(part 1 of 2)
# Autodesk Inventor assembly: enix_assembly_v2
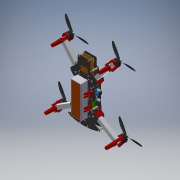
[picture p0: Inventor's stored thumbnail of the model, 180x180]
Saved by Autodesk Inventor 2016 (Build 200138000, 138)
## iProperties
Created: 2016-09-22
Part Number: enix_assembly_v2
Document SubType Name: Assembly
Designer: Jakub
Mass: 900.704 g
Surface Area: 2958.68 cm^2
Volume: 363.924 cm^3
Density: 2.47498 g/cm^3
Author: Jakub
## Documents named in this file (32)
- C:\Users\Jakub\Documents\DATA BANK\Projekty\Dron\Enix\V4\enix_assembly_v4.iam
- C:\Users\Jakub\Documents\DATA BANK\Projekty\Dron\Enix\V4\baseplate.ipt
- C:\Users\Jakub\Documents\DATA BANK\Projekty\Dron\Enix\V4\dist25mm.ipt
- C:\Users\Jakub\Documents\Inventor\Content Center Files\R2016\en-US\AS 1427(04)\AS 1427 - M2 x 8(5) I.ipt
- C:\Users\Jakub\Documents\Inventor\Content Center Files\R2016\en-US\AS 1112 (2)\AS 1112 - M2  Type 5.ipt
- C:\Users\Jakub\Documents\DATA BANK\Projekty\Dron\Enix\V4\top_plate.ipt
- C:\Users\Jakub\Documents\Inventor\Content Center Files\R2016\en-US\AS 1427(05)\AS 1427 - M3 x 5(5) II.ipt
- C:\Users\Jakub\Documents\DATA BANK\Projekty\Dron\Enix\V4\regulator.ipt
- C:\Users\Jakub\Documents\DATA BANK\Projekty\Dron\Enix\V4\dist10mmM2.ipt
- C:\Users\Jakub\Documents\DATA BANK\Projekty\Dron\Enix\V4\RASPBERRY PI 3.ipt
- C:\Users\Jakub\Documents\DATA BANK\Projekty\Dron\Enix\V4\dist5mmM2.ipt
- C:\Users\Jakub\Documents\DATA BANK\Projekty\Dron\Enix\V4\cam_holder.ipt
- C:\Users\Jakub\Documents\DATA BANK\Projekty\Dron\Enix\V4\arm_front_rect.ipt
- C:\Users\Jakub\Documents\DATA BANK\Projekty\Dron\Enix\V4\arm_back_rect.ipt
- C:\Users\Jakub\Documents\DATA BANK\Projekty\Dron\Enix\V4\motor_mount.ipt
- C:\Users\Jakub\Documents\DATA BANK\Projekty\Dron\Enix\V4\motor_mount_lock.ipt
- C:\Users\Jakub\Documents\DATA BANK\Projekty\Dron\Enix\V4\Emax Rs2205 v1.ipt
- C:\Users\Jakub\Documents\DATA BANK\Projekty\Dron\Enix\V4\5x3_prop.ipt
- C:\Users\Jakub\Documents\DATA BANK\Projekty\Dron\Enix\V4\logic_conventer_lock.ipt
- C:\Users\Jakub\Documents\DATA BANK\Projekty\Dron\Enix\V4\altimuv3.iam
- C:\Users\Jakub\Documents\DATA BANK\Projekty\Dron\Enix\V4\kamamiLogicVoltageConverter\converter.iam
- C:\Users\Jakub\Documents\DATA BANK\Projekty\Dron\Enix\V4\kamamiTransformer\transformer.iam
- C:\Users\Jakub\Documents\DATA BANK\Projekty\Dron\Enix\V4\battery_distancer.ipt
- C:\Users\Jakub\Documents\DATA BANK\Projekty\Dron\Enix\V4\battery_vant_4500_4s.ipt
- C:\Users\Jakub\Documents\DATA BANK\Projekty\Dron\Enix\V4\arm_socket_l.ipt
- C:\Users\Jakub\Documents\DATA BANK\Projekty\Dron\Enix\V4\arm_socket_r.ipt
- C:\Users\Jakub\Documents\Inventor\Content Center Files\R2016\en-US\AS 1427(04)\AS 1427 - M2 x 12(5) I.ipt
- C:\Users\Jakub\Documents\Inventor\Content Center Files\R2016\en-US\AS 1427(05)\AS 1427 - M3 x 10(5) II.ipt
- C:\Users\Jakub\Documents\Inventor\Content Center Files\R2016\en-US\ANSI B18.2.4.2M\ANSI B18.2.4.2M - M3x0,5 - 5,5.ipt
- C:\Users\Jakub\Documents\Inventor\Content Center Files\R2016\en-US\AS 1427(05)\AS 1427 - M3 x 30(5) II.ipt
- C:\Users\Jakub\Documents\DATA BANK\Projekty\Dron\Enix\V4\transformer_mount_new.ipt
- C:\Users\Jakub\Documents\DATA BANK\Projekty\Dron\Enix\V4\kamera.ipt
## Components (243 placed, 31 different names)
1. baseplate:1 — Mate:20, Mate:21, Mate:22, Mate:23, Mate:24, Mate:25, Mate:26, Mate:27, Mate:28, Mate:29, Mate:30, Mate:31, Mate:64, Mate:65, Mate:66, Mate:67, Mate:68, Mate:69, Mate:70, Mate:71, Mate:156, Mate:157, Mate:158, Mate:159, Mate:160, Mate:161, Mate:162, Mate:163, Mate:164, Mate:165, Mate:166, Mate:167, Mate:168, Mate:169, Mate:170, Mate:171, Mate:172, Mate:173, Mate:174, Mate:175, Mate:280, Mate:281, Mate:282, Mate:283, Mate:284, Mate:285, Mate:298, Mate:299, Mate:300, Mate:313, Mate:314, Mate:315, Mate:328, Mate:329, Mate:409, Mate:410, Mate:415, Mate:417, Mate:418, Mate:428, Mate:443, Mate:444, Mate:445, Mate:446, Mate:447, Mate:448, Mate:449, Mate:450, Mate:451, Mate:452, Mate:453, Mate:454, Mate:528, Mate:530, Mate:532, Mate:533, Mate:534, Mate:535, Mate:536, Mate:537, Mate:538, Mate:539, Mate:540, Mate:541, Mate:542, Mate:543, Mate:544, Mate:545, Mate:574, Mate:575, Angle:9, Mate:576, Mate:577, Angle:10, Mate:584, Mate:585, Angle:11, Mate:586, Mate:587, Angle:12, Mate:712, Mate:713, Mate:724, Mate:725, Mate:732, Mate:733, Mate:738, Mate:740, Mate:752, Mate:753, Mate:756, Mate:757, Mate:758, Mate:795, Mate:796, Mate:797, Mate:805, Mate:807, Mate:817, Mate:818, Mate:819, Mate:827, Mate:830
2. dist25mm:1 — Mate:20, Mate:23
3. dist25mm:2 — Mate:21, Mate:22
4. dist25mm:3 — Mate:27, Mate:28
5. dist25mm:4 — Mate:26, Mate:29
6. dist25mm:5 — Mate:25, Mate:30
7. dist25mm:6 — Mate:24, Mate:31, Mate:72, Mate:73
8. dist25mm:7 — Mate:68, Mate:69
9. dist25mm:8 — Mate:70, Mate:71, Mate:74
10. dist25mm:9 — Mate:66, Mate:67, Mate:75
11. dist25mm:10 — Mate:64, Mate:65
12. top_plate:1 — Mate:72, Mate:73, Mate:74, Mate:75, Mate:136, Mate:137, Mate:138, Mate:139, Mate:140, Mate:141, Mate:142, Mate:143, Mate:144, Mate:145, Mate:146, Mate:147, Mate:148, Mate:149, Mate:150, Mate:151, Mate:152, Mate:153, Mate:154, Mate:155, Mate:219, Mate:220, Mate:221, Mate:222, Mate:223, Mate:224, Mate:225, Mate:226, Mate:249, Mate:250, Mate:251, Mate:252, Mate:419, Mate:420, Mate:421, Mate:422, Mate:425, Mate:426, Mate:484, Mate:485, Mate:680, Mate:681, Mate:682, Mate:683, Mate:690, Mate:691, Mate:692, Mate:693, Mate:696, Mate:697, Mate:701, Mate:702, Mate:704, Mate:705, Mate:708, Mate:709, Mate:744, Mate:745, Mate:746, Mate:747, Mate:748, Mate:749, Mate:750, Mate:751
13. AS 1427 H - Metric M3 x 5:1 — Mate:137, Mate:145
14. AS 1427 H - Metric M3 x 5:2 — Mate:138, Mate:146
15. AS 1427 H - Metric M3 x 5:3 — Mate:154, Mate:155
16. AS 1427 H - Metric M3 x 5:4 — Mate:144, Mate:153
17. AS 1427 H - Metric M3 x 5:5 — Mate:143, Mate:151
18. AS 1427 H - Metric M3 x 5:6 — Mate:142, Mate:152
19. AS 1427 H - Metric M3 x 5:7 — Mate:141, Mate:149
20. AS 1427 H - Metric M3 x 5:8 — Mate:140, Mate:148
21. AS 1427 H - Metric M3 x 5:9 — Mate:139, Mate:147
22. AS 1427 H - Metric M3 x 5:10 — Mate:136, Mate:150
23. AS 1427 H - Metric M3 x 5:11 — Mate:165, Mate:166
24. AS 1427 H - Metric M3 x 5:12 — Mate:164, Mate:167
25. AS 1427 H - Metric M3 x 5:13 — Mate:163, Mate:168
26. AS 1427 H - Metric M3 x 5:14 — Mate:162, Mate:169
27. AS 1427 H - Metric M3 x 5:15 — Mate:161, Mate:170
28. AS 1427 H - Metric M3 x 5:16 — Mate:160, Mate:171
29. AS 1427 H - Metric M3 x 5:17 — Mate:159, Mate:172
30. AS 1427 H - Metric M3 x 5:18 — Mate:158, Mate:173
31. AS 1427 H - Metric M3 x 5:19 — Mate:157, Mate:175
32. AS 1427 H - Metric M3 x 5:20 — Mate:156, Mate:174
33. RASPBERRY PI 3:1 — Mate:227, Mate:228, Mate:229, Mate:230, Mate:243, Mate:244, Mate:245, Mate:246
34. dist5mmM2:2 — Mate:221, Mate:225, Mate:228, Mate:240, Mate:253
35. dist5mmM2:3 — Mate:220, Mate:226, Mate:227, Mate:229, Mate:241, Mate:256
36. dist5mmM2:4 — Mate:219, Mate:223, Mate:230, Mate:242, Mate:255
37. dist5mmM2:5 — Mate:222, Mate:224, Mate:239, Mate:254
38. AS 1427 H - Metric M2 x 8:17 — Mate:239, Mate:243
39. AS 1427 H - Metric M2 x 8:18 — Mate:240, Mate:244
40. AS 1427 H - Metric M2 x 8:19 — Mate:241, Mate:245
41. AS 1427 H - Metric M2 x 8:20 — Mate:242, Mate:246
42. AS 1112 (2) - Metric M2  Type 5:20 — Mate:249, Mate:253
43. AS 1112 (2) - Metric M2  Type 5:21 — Mate:250, Mate:254
44. AS 1112 (2) - Metric M2  Type 5:22 — Mate:251, Mate:256
45. AS 1112 (2) - Metric M2  Type 5:23 — Mate:252, Mate:255
46. dist5mmM2:6 — Mate:282, Mate:284, Mate:302, Mate:459
47. dist5mmM2:7 — Mate:281, Mate:283, Mate:301
48. dist5mmM2:8 — Mate:280, Mate:285, Mate:303
49. dist10mmM2:7
50. dist10mmM2:8
51. dist10mmM2:9 — Mate:461
52. AS 1112 (2) - Metric M2  Type 5:24 — Mate:298, Mate:302
53. AS 1112 (2) - Metric M2  Type 5:25 — Mate:300, Mate:303
54. AS 1112 (2) - Metric M2  Type 5:26 — Mate:299, Mate:301
55. AS 1427 H - Metric M2 x 8:21 — Mate:462
56. AS 1427 H - Metric M2 x 8:22
57. AS 1427 H - Metric M2 x 8:23
58. cam_holder:1 — Mate:313, Mate:314, Mate:315, Mate:316, Mate:317, Mate:318, Mate:319, Mate:332, Mate:333, Mate:334, Mate:335, Mate:839, Mate:840, Mate:841
59. AS 1427 H - Metric M2 x 8:24 — Mate:317, Mate:319, Mate:330
60. AS 1427 H - Metric M2 x 8:28 — Mate:316, Mate:318, Mate:331
61. AS 1112 (2) - Metric M2  Type 5:27 — Mate:329, Mate:330
62. AS 1112 (2) - Metric M2  Type 5:28 — Mate:328, Mate:331
63. AS 1112 (2) - Metric M2  Type 5:29 — Mate:332, Mate:852
64. AS 1112 (2) - Metric M2  Type 5:30 — Mate:333
65. AS 1112 (2) - Metric M2  Type 5:31 — Mate:334, Mate:851
66. AS 1112 (2) - Metric M2  Type 5:32 — Mate:335
67. arm_front_rect:1 — Mate:350, Mate:356, Angle:8, Mate:361, Mate:566, Mate:581, Mate:582, Mate:583, Angle:11, Mate:622
68. arm_front_rect:2 — Mate:351, Mate:357, Angle:7, Mate:358, Mate:565, Mate:571, Mate:572, Mate:573, Angle:10, Mate:634
69. arm_back_rect:1 — Mate:352, Mate:355, Angle:6, Mate:364, Mate:567, Mate:578, Mate:579, Mate:580, Angle:12, Mate:630
70. arm_back_rect:2 — Mate:353, Mate:354, Angle:5, Mate:367, Mate:564, Mate:568, Mate:569, Mate:570, Angle:9, Mate:632
71. motor_mount:1 — Mate:350, Mate:356, Angle:8, Mate:362, Mate:363, Mate:592, Mate:593, Mate:594, Mate:595, Mate:658, Mate:659, Mate:660, Mate:661, Mate:662, Mate:663, Mate:664, Mate:665, Mate:666
72. motor_mount:2 — Mate:351, Mate:357, Angle:7, Mate:359, Mate:360, Mate:588, Mate:589, Mate:590, Mate:591, Mate:669, Mate:670, Mate:671, Mate:672, Mate:673, Mate:674, Mate:675, Mate:676, Mate:677
73. motor_mount:3 — Mate:353, Mate:354, Angle:5, Mate:368, Mate:369, Mate:600, Mate:601, Mate:602, Mate:603, Mate:636, Mate:637, Mate:638, Mate:639, Mate:640, Mate:641, Mate:642, Mate:643, Mate:644, Mate:645, Mate:646
74. motor_mount:4 — Mate:352, Mate:355, Angle:6, Mate:365, Mate:366, Mate:596, Mate:597, Mate:598, Mate:599, Mate:647, Mate:648, Mate:649, Mate:650, Mate:651, Mate:652, Mate:653, Mate:654, Mate:655
75. motor_mount_lock:1 — Mate:358, Mate:359, Mate:360, Mate:565, Mate:612, Mate:613, Mate:614, Mate:615, Mate:628, Mate:629
76. motor_mount_lock:2 — Mate:361, Mate:362, Mate:363, Mate:566, Mate:616, Mate:617, Mate:618, Mate:619, Mate:620, Mate:621
77. motor_mount_lock:3 — Mate:364, Mate:365, Mate:366, Mate:567, Mate:604, Mate:605, Mate:606, Mate:607, Mate:624, Mate:625
78. motor_mount_lock:4 — Mate:367, Mate:368, Mate:369, Mate:564, Mate:608, Mate:609, Mate:610, Mate:611, Mate:626, Mate:627
79. Emax Rs2205 v1:1 — Mate:379, Mate:384, Mate:677, Mate:678, Mate:679
80. Emax Rs2205 v1:2 — Mate:378, Mate:382, Mate:666, Mate:667, Mate:668
81. Emax Rs2205 v1:3 — Mate:381, Mate:383, Mate:655, Mate:656, Mate:657
82. Emax Rs2205 v1:4 — Mate:380, Mate:385, Mate:636, Mate:637, Mate:638
83. 5x3_prop:1 — Mate:380, Mate:385
84. 5x3_prop:2 — Mate:379, Mate:384
85. 5x3_prop:3 — Mate:378, Mate:382
86. 5x3_prop:4 — Mate:381, Mate:383
87. dist5mmM2:9 — Mate:409, Mate:410, Mate:412, Mate:414, Mate:416
88. dist10mmM2:12 — Mate:412, Mate:460
89. AS 1427 H - Metric M2 x 8:30 — Mate:414
90. AS 1112 (2) - Metric M2  Type 5:34 — Mate:415, Mate:416
91. logic_conventer_lock:1 — Mate:417, Mate:418, Flush:1, Mate:429, Mate:524, Mate:525, Mate:526, Mate:527
92. altimuv3:1 [sub-assembly] — Mate:427, Mate:486, Mate:487, Mate:488, Mate:489, Mate:490, Mate:491
93. dist5mmM2:10 — Mate:419, Mate:421, Mate:424, Mate:484
94. dist5mmM2:11 — Mate:420, Mate:422, Mate:423, Mate:427, Mate:485, Mate:486, Mate:487
95. AS 1112 (2) - Metric M2  Type 5:35 — Mate:423, Mate:425
96. AS 1112 (2) - Metric M2  Type 5:36 — Mate:424, Mate:426
97. converter:1 [sub-assembly] — Mate:428, Flush:1, Mate:429
98. transformer:2 [sub-assembly] — Mate:798, Mate:799, Mate:800, Mate:809, Mate:810, Mate:811, Mate:812
99. dist5mmM2:12 — Mate:445, Mate:450, Mate:458
100. dist5mmM2:13 — Mate:443, Mate:447, Mate:456, Mate:464
101. dist5mmM2:14 — Mate:446, Mate:449, Mate:455
102. dist5mmM2:15 — Mate:444, Mate:448, Mate:457, Mate:463
103. AS 1112 (2) - Metric M2  Type 5:37 — Mate:454, Mate:455
104. AS 1112 (2) - Metric M2  Type 5:38 — Mate:453, Mate:457
105. AS 1112 (2) - Metric M2  Type 5:39 — Mate:452, Mate:458
106. AS 1112 (2) - Metric M2  Type 5:40 — Mate:451, Mate:456
107. regulator:1 — Mate:459, Mate:460
108. regulator:2 — Mate:461, Mate:462
109. regulator:3 — Mate:463, Mate:464, Mate:465, Mate:466, Mate:467, Mate:468, Mate:469, Mate:470, Mate:471, Mate:472
110. regulator:4 — Mate:473, Mate:474, Mate:475, Mate:476, Mate:477, Mate:478, Mate:479, Mate:480, Mate:481, Mate:482, Mate:483
111. dist10mmM2:13 — Mate:467, Mate:472
112. dist10mmM2:14 — Mate:466, Mate:470, Mate:474
113. dist10mmM2:15 — Mate:465, Mate:469, Mate:473, Mate:475
114. dist10mmM2:16 — Mate:468, Mate:471
115. AS 1427 H - Metric M2 x 8:31 — Mate:479, Mate:483
116. AS 1427 H - Metric M2 x 8:32 — Mate:476, Mate:481
117. AS 1427 H - Metric M2 x 8:33 — Mate:477, Mate:480
118. AS 1427 H - Metric M2 x 8:34 — Mate:478, Mate:482
119. AS 1427 H - Metric M2 x 8:35 — Mate:488, Mate:491
120. AS 1427 H - Metric M2 x 8:36 — Mate:489, Mate:490
121. AS 1427 H - Metric M2 x 8:45 — Mate:524, Mate:527, Mate:531
122. AS 1427 H - Metric M2 x 8:46 — Mate:525, Mate:526, Mate:529
123. AS 1112 (2) - Metric M2  Type 5:49 — Mate:530, Mate:531
124. AS 1112 (2) - Metric M2  Type 5:50 — Mate:528, Mate:529
125. battery_distancer:1 — Mate:532, Mate:533, Mate:534, Mate:548, Mate:550
126. battery_distancer:2 — Mate:535, Mate:536, Mate:537, Mate:546, Mate:552, Mate:554, Mate:555
127. AS 1427 H - Metric M2 x 8:47 — Mate:538, Mate:539, Mate:553
128. AS 1427 H - Metric M2 x 8:48 — Mate:540, Mate:541, Mate:551
129. AS 1427 H - Metric M2 x 8:49 — Mate:543, Mate:544, Mate:549
130. AS 1427 H - Metric M2 x 8:50 — Mate:542, Mate:545, Mate:547
131. AS 1112 (2) - Metric M2  Type 5:51 — Mate:552, Mate:553
132. AS 1112 (2) - Metric M2  Type 5:52 — Mate:550, Mate:551
133. AS 1112 (2) - Metric M2  Type 5:53 — Mate:548, Mate:549
134. AS 1112 (2) - Metric M2  Type 5:54 — Mate:546, Mate:547
135. battery_vant_4500_4s:1 — Mate:554, Mate:555
136. arm_socket_l:1 — Mate:568, Mate:569, Mate:570, Mate:574, Mate:575, Mate:684, Mate:685, Mate:706, Mate:707, Mate:728, Mate:730
137. arm_socket_l:2 — Mate:571, Mate:572, Mate:573, Mate:576, Mate:577, Mate:686, Mate:687, Mate:688, Mate:689, Mate:736, Mate:742
138. arm_socket_r:1 — Mate:578, Mate:579, Mate:580, Mate:586, Mate:587, Mate:698, Mate:699, Mate:700, Mate:703, Mate:716, Mate:718
139. arm_socket_r:2 — Mate:581, Mate:582, Mate:583, Mate:584, Mate:585, Mate:694, Mate:695, Mate:710, Mate:711, Mate:720, Mate:722
140. AS 1112 (2) - Metric M2  Type 5:55 — Mate:588, Mate:589
141. AS 1112 (2) - Metric M2  Type 5:56 — Mate:590, Mate:591
142. AS 1112 (2) - Metric M2  Type 5:57 — Mate:600, Mate:601
143. AS 1112 (2) - Metric M2  Type 5:58 — Mate:602, Mate:603
144. AS 1112 (2) - Metric M2  Type 5:59 — Mate:598, Mate:599
145. AS 1112 (2) - Metric M2  Type 5:60 — Mate:596, Mate:597
146. AS 1112 (2) - Metric M2  Type 5:61 — Mate:592, Mate:593
147. AS 1112 (2) - Metric M2  Type 5:62 — Mate:594, Mate:595
148. AS 1427 H - Metric M2 x 12:2 — Mate:606, Mate:607
149. AS 1427 H - Metric M2 x 12:1 — Mate:604, Mate:605
150. AS 1427 H - Metric M2 x 12:3 — Mate:616, Mate:617
151. AS 1427 H - Metric M2 x 12:4 — Mate:618, Mate:619
152. AS 1427 H - Metric M2 x 12:5 — Mate:608, Mate:609
153. AS 1427 H - Metric M2 x 12:6 — Mate:610, Mate:611
154. AS 1427 H - Metric M2 x 12:7 — Mate:614, Mate:615
155. AS 1427 H - Metric M2 x 12:8 — Mate:612, Mate:613
156. AS 1427 H - Metric M3 x 10:1 — Mate:620, Mate:621, Mate:623
157. ANSI B18.2.4.2M M3x0,5:1 — Mate:622, Mate:623
158. AS 1427 H - Metric M3 x 10:2 — Mate:624, Mate:625, Mate:631
159. AS 1427 H - Metric M3 x 10:3 — Mate:626, Mate:627, Mate:633
160. AS 1427 H - Metric M3 x 10:4 — Mate:628, Mate:629, Mate:635
161. ANSI B18.2.4.2M M3x0,5:2 — Mate:630, Mate:631
162. ANSI B18.2.4.2M M3x0,5:3 — Mate:632, Mate:633
163. ANSI B18.2.4.2M M3x0,5:4 — Mate:634, Mate:635
164. AS 1427 H - Metric M3 x 5:21 — Mate:639, Mate:640
165. AS 1427 H - Metric M3 x 5:22 — Mate:645, Mate:646
166. AS 1427 H - Metric M3 x 5:23 — Mate:643, Mate:644
167. AS 1427 H - Metric M3 x 5:24 — Mate:641, Mate:642
168. AS 1427 H - Metric M3 x 5:25 — Mate:660, Mate:664
169. AS 1427 H - Metric M3 x 5:26 — Mate:659, Mate:663, Mate:667
170. AS 1427 H - Metric M3 x 5:27 — Mate:658, Mate:662, Mate:668
171. AS 1427 H - Metric M3 x 5:28 — Mate:661, Mate:665
172. AS 1427 H - Metric M3 x 5:29 — Mate:671, Mate:675, Mate:679
173. AS 1427 H - Metric M3 x 5:30 — Mate:672, Mate:673
174. AS 1427 H - Metric M3 x 5:31 — Mate:669, Mate:674
175. AS 1427 H - Metric M3 x 5:32 — Mate:670, Mate:676, Mate:678
176. AS 1427 H - Metric M3 x 5:33 — Mate:647, Mate:648, Mate:656
177. AS 1427 H - Metric M3 x 5:34 — Mate:649, Mate:650, Mate:657
178. AS 1427 H - Metric M3 x 5:35 — Mate:651, Mate:652
179. AS 1427 H - Metric M3 x 5:36 — Mate:653, Mate:654
180. AS 1427 H - Metric M2 x 8:55 — Mate:680, Mate:690, Mate:737
181. AS 1427 H - Metric M2 x 8:56 — Mate:682, Mate:705, Mate:729
182. AS 1427 H - Metric M2 x 8:57 — Mate:681, Mate:691, Mate:743
183. AS 1427 H - Metric M2 x 8:58 — Mate:684, Mate:706, Mate:735
184. AS 1427 H - Metric M2 x 8:59 — Mate:683, Mate:704, Mate:731
185. AS 1427 H - Metric M2 x 8:60 — Mate:685, Mate:707, Mate:734
186. AS 1427 H - Metric M2 x 8:61 — Mate:687, Mate:688, Mate:741
187. AS 1427 H - Metric M2 x 8:62 — Mate:686, Mate:689, Mate:739
188. AS 1427 H - Metric M2 x 8:63 — Mate:699, Mate:703, Mate:714
189. AS 1427 H - Metric M2 x 8:64 — Mate:698, Mate:700, Mate:715
190. AS 1427 H - Metric M2 x 8:65 — Mate:697, Mate:702, Mate:719
191. AS 1427 H - Metric M2 x 8:66 — Mate:696, Mate:701, Mate:717
192. AS 1427 H - Metric M2 x 8:67 — Mate:695, Mate:711, Mate:726
193. AS 1427 H - Metric M2 x 8:68 — Mate:694, Mate:710, Mate:727
194. AS 1427 H - Metric M2 x 8:69 — Mate:692, Mate:709, Mate:721
195. AS 1427 H - Metric M2 x 8:70 — Mate:693, Mate:708, Mate:723
196. AS 1112 (2) - Metric M2  Type 5:63 — Mate:718, Mate:719
197. AS 1112 (2) - Metric M2  Type 5:64 — Mate:716, Mate:717
198. AS 1112 (2) - Metric M2  Type 5:65 — Mate:713, Mate:714
199. AS 1112 (2) - Metric M2  Type 5:66 — Mate:712, Mate:715
200. AS 1112 (2) - Metric M2  Type 5:67 — Mate:720, Mate:721
201. AS 1112 (2) - Metric M2  Type 5:68 — Mate:725, Mate:726
202. AS 1112 (2) - Metric M2  Type 5:69 — Mate:724, Mate:727
203. AS 1112 (2) - Metric M2  Type 5:70 — Mate:722, Mate:723
204. AS 1112 (2) - Metric M2  Type 5:71 — Mate:736, Mate:737
205. AS 1112 (2) - Metric M2  Type 5:72 — Mate:738, Mate:739
206. AS 1112 (2) - Metric M2  Type 5:73 — Mate:742, Mate:743
207. AS 1112 (2) - Metric M2  Type 5:74 — Mate:740, Mate:741
208. AS 1112 (2) - Metric M2  Type 5:75 — Mate:730, Mate:731
209. AS 1112 (2) - Metric M2  Type 5:76 — Mate:733, Mate:734
210. AS 1112 (2) - Metric M2  Type 5:77 — Mate:728, Mate:729
211. AS 1112 (2) - Metric M2  Type 5:78 — Mate:732, Mate:735
212. AS 1427 H - Metric M3 x 30:1 — Mate:744, Mate:745, Mate:755
213. AS 1427 H - Metric M3 x 30:2 — Mate:746, Mate:751, Mate:754
214. AS 1427 H - Metric M3 x 30:3 — Mate:748, Mate:749
215. AS 1427 H - Metric M3 x 30:4 — Mate:747, Mate:750, Mate:759
216. ANSI B18.2.4.2M M3x0,5:5 — Mate:756, Mate:757
217. ANSI B18.2.4.2M M3x0,5:6 — Mate:753, Mate:754
218. ANSI B18.2.4.2M M3x0,5:7 — Mate:758, Mate:759
219. ANSI B18.2.4.2M M3x0,5:8 — Mate:752, Mate:755
220. transformer_mount_new:1 — Mate:795, Mate:796, Mate:797, Mate:798, Mate:799, Mate:800, Mate:801, Mate:802, Mate:803, Mate:804, Mate:813, Mate:815
221. AS 1427 H - Metric M2 x 8:77 — Mate:801, Mate:802, Mate:806
222. AS 1427 H - Metric M2 x 8:78 — Mate:803, Mate:804, Mate:808
223. AS 1112 (2) - Metric M2  Type 5:85 — Mate:805, Mate:806
224. AS 1112 (2) - Metric M2  Type 5:86 — Mate:807, Mate:808
225. AS 1427 H - Metric M2 x 8:79 — Mate:809, Mate:810, Mate:814
226. AS 1427 H - Metric M2 x 8:80 — Mate:811, Mate:812, Mate:816
227. AS 1112 (2) - Metric M2  Type 5:87 — Mate:813, Mate:814
228. AS 1112 (2) - Metric M2  Type 5:88 — Mate:815, Mate:816
229. transformer_mount_new:2 — Mate:817, Mate:818, Mate:819, Mate:820, Mate:821, Mate:822, Mate:825, Mate:826, Mate:828, Mate:829, Mate:835, Mate:837
230. transformer:3 [sub-assembly] — Mate:820, Mate:821, Mate:822, Mate:831, Mate:832, Mate:833, Mate:834
231. AS 1427 H - Metric M2 x 8:81 — Mate:825, Mate:826
232. AS 1112 (2) - Metric M2  Type 5:89 — Mate:827
233. AS 1427 H - Metric M2 x 8:82 — Mate:828, Mate:829
234. AS 1112 (2) - Metric M2  Type 5:90 — Mate:830
235. AS 1427 H - Metric M2 x 8:83 — Mate:831, Mate:832, Mate:838
236. AS 1427 H - Metric M2 x 8:84 — Mate:833, Mate:834, Mate:836
237. AS 1112 (2) - Metric M2  Type 5:91 — Mate:835, Mate:836
238. AS 1112 (2) - Metric M2  Type 5:92 — Mate:837, Mate:838
239. kamera:1 — Mate:839, Mate:840, Mate:841, Mate:842, Mate:844, Mate:845, Mate:846, Mate:847, Mate:848, Mate:849, Mate:850
240. AS 1427 H - Metric M2 x 8:85 — Mate:842, Mate:850
241. AS 1427 H - Metric M2 x 8:86 — Mate:845, Mate:849, Mate:851
242. AS 1427 H - Metric M2 x 8:87 — Mate:844, Mate:847
243. AS 1427 H - Metric M2 x 8:88 — Mate:846, Mate:848, Mate:852
## Relationships (509: Mate 500, Angle 8, Flush 1)
- Mate:20: baseplate:1 ↔ dist25mm:1
- Mate:21: baseplate:1 ↔ dist25mm:2
- Mate:22: baseplate:1 ↔ dist25mm:2
- Mate:23: baseplate:1 ↔ dist25mm:1
- Mate:24: baseplate:1 ↔ dist25mm:6
- Mate:25: baseplate:1 ↔ dist25mm:5
- Mate:26: baseplate:1 ↔ dist25mm:4
- Mate:27: baseplate:1 ↔ dist25mm:3
- Mate:28: baseplate:1 ↔ dist25mm:3
- Mate:29: baseplate:1 ↔ dist25mm:4
- Mate:30: baseplate:1 ↔ dist25mm:5
- Mate:31: baseplate:1 ↔ dist25mm:6
- Mate:64: baseplate:1 ↔ dist25mm:10
- Mate:65: baseplate:1 ↔ dist25mm:10
- Mate:66: baseplate:1 ↔ dist25mm:9
- Mate:67: baseplate:1 ↔ dist25mm:9
- Mate:68: baseplate:1 ↔ dist25mm:7
- Mate:69: baseplate:1 ↔ dist25mm:7
- Mate:70: baseplate:1 ↔ dist25mm:8
- Mate:71: baseplate:1 ↔ dist25mm:8
- Mate:72: dist25mm:6 ↔ top_plate:1
- Mate:73: dist25mm:6 ↔ top_plate:1
- Mate:74: dist25mm:8 ↔ top_plate:1
- Mate:75: dist25mm:9 ↔ top_plate:1
- Mate:136: top_plate:1 ↔ AS 1427 H - Metric M3 x 5:10
- Mate:137: top_plate:1 ↔ AS 1427 H - Metric M3 x 5:1
- Mate:138: top_plate:1 ↔ AS 1427 H - Metric M3 x 5:2
- Mate:139: top_plate:1 ↔ AS 1427 H - Metric M3 x 5:9
- Mate:140: top_plate:1 ↔ AS 1427 H - Metric M3 x 5:8
- Mate:141: top_plate:1 ↔ AS 1427 H - Metric M3 x 5:7
- Mate:142: top_plate:1 ↔ AS 1427 H - Metric M3 x 5:6
- Mate:143: top_plate:1 ↔ AS 1427 H - Metric M3 x 5:5
- Mate:144: top_plate:1 ↔ AS 1427 H - Metric M3 x 5:4
- Mate:145: top_plate:1 ↔ AS 1427 H - Metric M3 x 5:1
- Mate:146: top_plate:1 ↔ AS 1427 H - Metric M3 x 5:2
- Mate:147: top_plate:1 ↔ AS 1427 H - Metric M3 x 5:9
- Mate:148: top_plate:1 ↔ AS 1427 H - Metric M3 x 5:8
- Mate:149: top_plate:1 ↔ AS 1427 H - Metric M3 x 5:7
- Mate:150: top_plate:1 ↔ AS 1427 H - Metric M3 x 5:10
- Mate:151: top_plate:1 ↔ AS 1427 H - Metric M3 x 5:5
- Mate:152: top_plate:1 ↔ AS 1427 H - Metric M3 x 5:6
- Mate:153: top_plate:1 ↔ AS 1427 H - Metric M3 x 5:4
- Mate:154: top_plate:1 ↔ AS 1427 H - Metric M3 x 5:3
- Mate:155: top_plate:1 ↔ AS 1427 H - Metric M3 x 5:3
- Mate:156: baseplate:1 ↔ AS 1427 H - Metric M3 x 5:20
- Mate:157: baseplate:1 ↔ AS 1427 H - Metric M3 x 5:19
- Mate:158: baseplate:1 ↔ AS 1427 H - Metric M3 x 5:18
- Mate:159: baseplate:1 ↔ AS 1427 H - Metric M3 x 5:17
- Mate:160: baseplate:1 ↔ AS 1427 H - Metric M3 x 5:16
- Mate:161: baseplate:1 ↔ AS 1427 H - Metric M3 x 5:15
- Mate:162: baseplate:1 ↔ AS 1427 H - Metric M3 x 5:14
- Mate:163: baseplate:1 ↔ AS 1427 H - Metric M3 x 5:13
- Mate:164: baseplate:1 ↔ AS 1427 H - Metric M3 x 5:12
- Mate:165: baseplate:1 ↔ AS 1427 H - Metric M3 x 5:11
- Mate:166: baseplate:1 ↔ AS 1427 H - Metric M3 x 5:11
- Mate:167: baseplate:1 ↔ AS 1427 H - Metric M3 x 5:12
- Mate:168: baseplate:1 ↔ AS 1427 H - Metric M3 x 5:13
- Mate:169: baseplate:1 ↔ AS 1427 H - Metric M3 x 5:14
- Mate:170: baseplate:1 ↔ AS 1427 H - Metric M3 x 5:15
- Mate:171: baseplate:1 ↔ AS 1427 H - Metric M3 x 5:16
- Mate:172: baseplate:1 ↔ AS 1427 H - Metric M3 x 5:17
- Mate:173: baseplate:1 ↔ AS 1427 H - Metric M3 x 5:18
- Mate:174: baseplate:1 ↔ AS 1427 H - Metric M3 x 5:20
- Mate:175: baseplate:1 ↔ AS 1427 H - Metric M3 x 5:19
- Mate:219: top_plate:1 ↔ dist5mmM2:4
- Mate:220: top_plate:1 ↔ dist5mmM2:3
- Mate:221: top_plate:1 ↔ dist5mmM2:2
- Mate:222: top_plate:1 ↔ dist5mmM2:5
- Mate:223: top_plate:1 ↔ dist5mmM2:4
- Mate:224: top_plate:1 ↔ dist5mmM2:5
- Mate:225: top_plate:1 ↔ dist5mmM2:2
- Mate:226: top_plate:1 ↔ dist5mmM2:3
- Mate:227: RASPBERRY PI 3:1 ↔ dist5mmM2:3
- Mate:228: RASPBERRY PI 3:1 ↔ dist5mmM2:2
- Mate:229: RASPBERRY PI 3:1 ↔ dist5mmM2:3
- Mate:230: RASPBERRY PI 3:1 ↔ dist5mmM2:4
- Mate:239: dist5mmM2:5 ↔ AS 1427 H - Metric M2 x 8:17
- Mate:240: dist5mmM2:2 ↔ AS 1427 H - Metric M2 x 8:18
- Mate:241: dist5mmM2:3 ↔ AS 1427 H - Metric M2 x 8:19
- Mate:242: dist5mmM2:4 ↔ AS 1427 H - Metric M2 x 8:20
- Mate:243: RASPBERRY PI 3:1 ↔ AS 1427 H - Metric M2 x 8:17
- Mate:244: RASPBERRY PI 3:1 ↔ AS 1427 H - Metric M2 x 8:18
- Mate:245: RASPBERRY PI 3:1 ↔ AS 1427 H - Metric M2 x 8:19
- Mate:246: RASPBERRY PI 3:1 ↔ AS 1427 H - Metric M2 x 8:20
- Mate:249: top_plate:1 ↔ AS 1112 (2) - Metric M2  Type 5:20
- Mate:250: top_plate:1 ↔ AS 1112 (2) - Metric M2  Type 5:21
- Mate:251: top_plate:1 ↔ AS 1112 (2) - Metric M2  Type 5:22
- Mate:252: top_plate:1 ↔ AS 1112 (2) - Metric M2  Type 5:23
- Mate:253: dist5mmM2:2 ↔ AS 1112 (2) - Metric M2  Type 5:20
- Mate:254: dist5mmM2:5 ↔ AS 1112 (2) - Metric M2  Type 5:21
- Mate:255: dist5mmM2:4 ↔ AS 1112 (2) - Metric M2  Type 5:23
- Mate:256: dist5mmM2:3 ↔ AS 1112 (2) - Metric M2  Type 5:22
- Mate:280: baseplate:1 ↔ dist5mmM2:8
- Mate:281: baseplate:1 ↔ dist5mmM2:7
- Mate:282: baseplate:1 ↔ dist5mmM2:6
- Mate:283: baseplate:1 ↔ dist5mmM2:7
- Mate:284: baseplate:1 ↔ dist5mmM2:6
- Mate:285: baseplate:1 ↔ dist5mmM2:8
- Mate:298: baseplate:1 ↔ AS 1112 (2) - Metric M2  Type 5:24
- Mate:299: baseplate:1 ↔ AS 1112 (2) - Metric M2  Type 5:26
- Mate:300: baseplate:1 ↔ AS 1112 (2) - Metric M2  Type 5:25
- Mate:301: dist5mmM2:7 ↔ AS 1112 (2) - Metric M2  Type 5:26
- Mate:302: dist5mmM2:6 ↔ AS 1112 (2) - Metric M2  Type 5:24
- Mate:303: dist5mmM2:8 ↔ AS 1112 (2) - Metric M2  Type 5:25
- Mate:313: baseplate:1 ↔ cam_holder:1
- Mate:314: baseplate:1 ↔ cam_holder:1
- Mate:315: baseplate:1 ↔ cam_holder:1
- Mate:316: cam_holder:1 ↔ AS 1427 H - Metric M2 x 8:28
- Mate:317: cam_holder:1 ↔ AS 1427 H - Metric M2 x 8:24
- Mate:318: cam_holder:1 ↔ AS 1427 H - Metric M2 x 8:28
- Mate:319: cam_holder:1 ↔ AS 1427 H - Metric M2 x 8:24
- Mate:328: baseplate:1 ↔ AS 1112 (2) - Metric M2  Type 5:28
- Mate:329: baseplate:1 ↔ AS 1112 (2) - Metric M2  Type 5:27
- Mate:330: AS 1427 H - Metric M2 x 8:24 ↔ AS 1112 (2) - Metric M2  Type 5:27
- Mate:331: AS 1427 H - Metric M2 x 8:28 ↔ AS 1112 (2) - Metric M2  Type 5:28
- Mate:332: cam_holder:1 ↔ AS 1112 (2) - Metric M2  Type 5:29
- Mate:333: cam_holder:1 ↔ AS 1112 (2) - Metric M2  Type 5:30
- Mate:334: cam_holder:1 ↔ AS 1112 (2) - Metric M2  Type 5:31
- Mate:335: cam_holder:1 ↔ AS 1112 (2) - Metric M2  Type 5:32
- Mate:350: arm_front_rect:1 ↔ motor_mount:1
- Mate:351: arm_front_rect:2 ↔ motor_mount:2
- Mate:352: arm_back_rect:1 ↔ motor_mount:4
- Mate:353: arm_back_rect:2 ↔ motor_mount:3
- Mate:354: arm_back_rect:2 ↔ motor_mount:3
- Mate:355: arm_back_rect:1 ↔ motor_mount:4
- Mate:356: arm_front_rect:1 ↔ motor_mount:1
- Mate:357: arm_front_rect:2 ↔ motor_mount:2
- Angle:5 (0 deg): arm_back_rect:2 ↔ motor_mount:3
- Angle:6 (0 deg): arm_back_rect:1 ↔ motor_mount:4
- Angle:7 (0 deg): arm_front_rect:2 ↔ motor_mount:2
- Angle:8 (0 deg): arm_front_rect:1 ↔ motor_mount:1
- Mate:358: arm_front_rect:2 ↔ motor_mount_lock:1
- Mate:359: motor_mount:2 ↔ motor_mount_lock:1
- Mate:360: motor_mount:2 ↔ motor_mount_lock:1
- Mate:361: arm_front_rect:1 ↔ motor_mount_lock:2
- Mate:362: motor_mount:1 ↔ motor_mount_lock:2
- Mate:363: motor_mount:1 ↔ motor_mount_lock:2
- Mate:364: arm_back_rect:1 ↔ motor_mount_lock:3
- Mate:365: motor_mount:4 ↔ motor_mount_lock:3
- Mate:366: motor_mount:4 ↔ motor_mount_lock:3
- Mate:367: arm_back_rect:2 ↔ motor_mount_lock:4
- Mate:368: motor_mount:3 ↔ motor_mount_lock:4
- Mate:369: motor_mount:3 ↔ motor_mount_lock:4
- Mate:378: Emax Rs2205 v1:2 ↔ 5x3_prop:3
- Mate:379: Emax Rs2205 v1:1 ↔ 5x3_prop:2
- Mate:380: Emax Rs2205 v1:4 ↔ 5x3_prop:1
- Mate:381: Emax Rs2205 v1:3 ↔ 5x3_prop:4
- Mate:382 (5 mm): Emax Rs2205 v1:2 ↔ 5x3_prop:3
- Mate:383 (5 mm): Emax Rs2205 v1:3 ↔ 5x3_prop:4
- Mate:384 (5 mm): Emax Rs2205 v1:1 ↔ 5x3_prop:2
- Mate:385 (5 mm): Emax Rs2205 v1:4 ↔ 5x3_prop:1
- Mate:409: baseplate:1 ↔ dist5mmM2:9
- Mate:410: baseplate:1 ↔ dist5mmM2:9
- Mate:412: dist5mmM2:9 ↔ dist10mmM2:12
- Mate:414: dist5mmM2:9 ↔ AS 1427 H - Metric M2 x 8:30
- Mate:415: baseplate:1 ↔ AS 1112 (2) - Metric M2  Type 5:34
- Mate:416: dist5mmM2:9 ↔ AS 1112 (2) - Metric M2  Type 5:34
- Mate:417: baseplate:1 ↔ logic_conventer_lock:1
- Mate:418: baseplate:1 ↔ logic_conventer_lock:1
- Mate:419: top_plate:1 ↔ dist5mmM2:10
- Mate:420: top_plate:1 ↔ dist5mmM2:11
- Mate:421: top_plate:1 ↔ dist5mmM2:10
- Mate:422: top_plate:1 ↔ dist5mmM2:11
- Mate:423: dist5mmM2:11 ↔ AS 1112 (2) - Metric M2  Type 5:35
- Mate:424: dist5mmM2:10 ↔ AS 1112 (2) - Metric M2  Type 5:36
- Mate:425: top_plate:1 ↔ AS 1112 (2) - Metric M2  Type 5:35
- Mate:426: top_plate:1 ↔ AS 1112 (2) - Metric M2  Type 5:36
- Mate:427: altimuv3:1 ↔ dist5mmM2:11
- Mate:428: baseplate:1 ↔ converter:1
- Flush:1: logic_conventer_lock:1 ↔ converter:1
- Mate:429: logic_conventer_lock:1 ↔ converter:1
- Mate:443: baseplate:1 ↔ dist5mmM2:13
- Mate:444: baseplate:1 ↔ dist5mmM2:15
- Mate:445: baseplate:1 ↔ dist5mmM2:12
- Mate:446: baseplate:1 ↔ dist5mmM2:14
- Mate:447: baseplate:1 ↔ dist5mmM2:13
- Mate:448: baseplate:1 ↔ dist5mmM2:15
- Mate:449: baseplate:1 ↔ dist5mmM2:14
- Mate:450: baseplate:1 ↔ dist5mmM2:12
- Mate:451: baseplate:1 ↔ AS 1112 (2) - Metric M2  Type 5:40
- Mate:452: baseplate:1 ↔ AS 1112 (2) - Metric M2  Type 5:39
- Mate:453: baseplate:1 ↔ AS 1112 (2) - Metric M2  Type 5:38
- Mate:454: baseplate:1 ↔ AS 1112 (2) - Metric M2  Type 5:37
- Mate:455: dist5mmM2:14 ↔ AS 1112 (2) - Metric M2  Type 5:37
- Mate:456: dist5mmM2:13 ↔ AS 1112 (2) - Metric M2  Type 5:40
- Mate:457: dist5mmM2:15 ↔ AS 1112 (2) - Metric M2  Type 5:38
- Mate:458: dist5mmM2:12 ↔ AS 1112 (2) - Metric M2  Type 5:39
- Mate:459: dist5mmM2:6 ↔ regulator:1
- Mate:460: dist10mmM2:12 ↔ regulator:1
- Mate:461: dist10mmM2:9 ↔ regulator:2
- Mate:462: AS 1427 H - Metric M2 x 8:21 ↔ regulator:2
- Mate:463: dist5mmM2:15 ↔ regulator:3
- Mate:464: dist5mmM2:13 ↔ regulator:3
- Mate:465: regulator:3 ↔ dist10mmM2:15
- Mate:466: regulator:3 ↔ dist10mmM2:14
- Mate:467: regulator:3 ↔ dist10mmM2:13
- Mate:468: regulator:3 ↔ dist10mmM2:16
- Mate:469: regulator:3 ↔ dist10mmM2:15
- Mate:470: regulator:3 ↔ dist10mmM2:14
- Mate:471: regulator:3 ↔ dist10mmM2:16
- Mate:472: regulator:3 ↔ dist10mmM2:13
- Mate:473: regulator:4 ↔ dist10mmM2:15
- Mate:474: regulator:4 ↔ dist10mmM2:14
- Mate:475: regulator:4 ↔ dist10mmM2:15
- Mate:476: regulator:4 ↔ AS 1427 H - Metric M2 x 8:32
- Mate:477: regulator:4 ↔ AS 1427 H - Metric M2 x 8:33
- Mate:478: regulator:4 ↔ AS 1427 H - Metric M2 x 8:34
- Mate:479: regulator:4 ↔ AS 1427 H - Metric M2 x 8:31
- Mate:480: regulator:4 ↔ AS 1427 H - Metric M2 x 8:33
- Mate:481: regulator:4 ↔ AS 1427 H - Metric M2 x 8:32
- Mate:482: regulator:4 ↔ AS 1427 H - Metric M2 x 8:34
- Mate:483: regulator:4 ↔ AS 1427 H - Metric M2 x 8:31
- Mate:484: top_plate:1 ↔ dist5mmM2:10
- Mate:485: top_plate:1 ↔ dist5mmM2:11
- Mate:486: altimuv3:1 ↔ dist5mmM2:11
- Mate:487: altimuv3:1 ↔ dist5mmM2:11
- Mate:488: altimuv3:1 ↔ AS 1427 H - Metric M2 x 8:35
- Mate:489: altimuv3:1 ↔ AS 1427 H - Metric M2 x 8:36
- Mate:490: altimuv3:1 ↔ AS 1427 H - Metric M2 x 8:36
- Mate:491: altimuv3:1 ↔ AS 1427 H - Metric M2 x 8:35
- Mate:524: logic_conventer_lock:1 ↔ AS 1427 H - Metric M2 x 8:45
- Mate:525: logic_conventer_lock:1 ↔ AS 1427 H - Metric M2 x 8:46
- Mate:526: logic_conventer_lock:1 ↔ AS 1427 H - Metric M2 x 8:46
- Mate:527: logic_conventer_lock:1 ↔ AS 1427 H - Metric M2 x 8:45
- Mate:528: baseplate:1 ↔ AS 1112 (2) - Metric M2  Type 5:50
- Mate:529: AS 1427 H - Metric M2 x 8:46 ↔ AS 1112 (2) - Metric M2  Type 5:50
- Mate:530: baseplate:1 ↔ AS 1112 (2) - Metric M2  Type 5:49
- Mate:531: AS 1427 H - Metric M2 x 8:45 ↔ AS 1112 (2) - Metric M2  Type 5:49
- Mate:532: baseplate:1 ↔ battery_distancer:1
- Mate:533: baseplate:1 ↔ battery_distancer:1
- Mate:534: baseplate:1 ↔ battery_distancer:1
- Mate:535: baseplate:1 ↔ battery_distancer:2
- Mate:536: baseplate:1 ↔ battery_distancer:2
- Mate:537: baseplate:1 ↔ battery_distancer:2
- Mate:538: baseplate:1 ↔ AS 1427 H - Metric M2 x 8:47
- Mate:539: baseplate:1 ↔ AS 1427 H - Metric M2 x 8:47
- Mate:540: baseplate:1 ↔ AS 1427 H - Metric M2 x 8:48
- Mate:541: baseplate:1 ↔ AS 1427 H - Metric M2 x 8:48
- Mate:542: baseplate:1 ↔ AS 1427 H - Metric M2 x 8:50
- Mate:543: baseplate:1 ↔ AS 1427 H - Metric M2 x 8:49
- Mate:544: baseplate:1 ↔ AS 1427 H - Metric M2 x 8:49
- Mate:545: baseplate:1 ↔ AS 1427 H - Metric M2 x 8:50
- Mate:546: battery_distancer:2 ↔ AS 1112 (2) - Metric M2  Type 5:54
- Mate:547: AS 1427 H - Metric M2 x 8:50 ↔ AS 1112 (2) - Metric M2  Type 5:54
- Mate:548: battery_distancer:1 ↔ AS 1112 (2) - Metric M2  Type 5:53
- Mate:549: AS 1427 H - Metric M2 x 8:49 ↔ AS 1112 (2) - Metric M2  Type 5:53
- Mate:550: battery_distancer:1 ↔ AS 1112 (2) - Metric M2  Type 5:52
- Mate:551: AS 1427 H - Metric M2 x 8:48 ↔ AS 1112 (2) - Metric M2  Type 5:52
- Mate:552: battery_distancer:2 ↔ AS 1112 (2) - Metric M2  Type 5:51
- Mate:553: AS 1427 H - Metric M2 x 8:47 ↔ AS 1112 (2) - Metric M2  Type 5:51
- Mate:554: battery_distancer:2 ↔ battery_vant_4500_4s:1
- Mate:555 (1 mm): battery_distancer:2 ↔ battery_vant_4500_4s:1
- Mate:564: arm_back_rect:2 ↔ motor_mount_lock:4
- Mate:565: arm_front_rect:2 ↔ motor_mount_lock:1
- Mate:566: arm_front_rect:1 ↔ motor_mount_lock:2
- Mate:567: arm_back_rect:1 ↔ motor_mount_lock:3
- Mate:568: arm_back_rect:2 ↔ arm_socket_l:1
- Mate:569: arm_back_rect:2 ↔ arm_socket_l:1
- Mate:570 (0.05 mm): arm_back_rect:2 ↔ arm_socket_l:1
- Mate:571: arm_front_rect:2 ↔ arm_socket_l:2
- Mate:572: arm_front_rect:2 ↔ arm_socket_l:2
- Mate:573 (0.05 mm): arm_front_rect:2 ↔ arm_socket_l:2
- Mate:574: baseplate:1 ↔ arm_socket_l:1
- Mate:575: baseplate:1 ↔ arm_socket_l:1
- Angle:9 (0 deg): baseplate:1 ↔ arm_back_rect:2
- Mate:576: baseplate:1 ↔ arm_socket_l:2
- Mate:577: baseplate:1 ↔ arm_socket_l:2
- Angle:10 (0 deg): baseplate:1 ↔ arm_front_rect:2
- Mate:578: arm_back_rect:1 ↔ arm_socket_r:1
- Mate:579 (0.05 mm): arm_back_rect:1 ↔ arm_socket_r:1
- Mate:580: arm_back_rect:1 ↔ arm_socket_r:1
- Mate:581: arm_front_rect:1 ↔ arm_socket_r:2
- Mate:582 (0.05 mm): arm_front_rect:1 ↔ arm_socket_r:2
- Mate:583: arm_front_rect:1 ↔ arm_socket_r:2
- Mate:584: baseplate:1 ↔ arm_socket_r:2
- Mate:585: baseplate:1 ↔ arm_socket_r:2
- Angle:11 (0 deg): baseplate:1 ↔ arm_front_rect:1
- Mate:586: baseplate:1 ↔ arm_socket_r:1
- Mate:587: baseplate:1 ↔ arm_socket_r:1
- Angle:12 (0 deg): baseplate:1 ↔ arm_back_rect:1
- Mate:588: motor_mount:2 ↔ AS 1112 (2) - Metric M2  Type 5:55
- Mate:589: motor_mount:2 ↔ AS 1112 (2) - Metric M2  Type 5:55
- Mate:590: motor_mount:2 ↔ AS 1112 (2) - Metric M2  Type 5:56
- Mate:591: motor_mount:2 ↔ AS 1112 (2) - Metric M2  Type 5:56
- Mate:592: motor_mount:1 ↔ AS 1112 (2) - Metric M2  Type 5:61
- Mate:593: motor_mount:1 ↔ AS 1112 (2) - Metric M2  Type 5:61
- Mate:594: motor_mount:1 ↔ AS 1112 (2) - Metric M2  Type 5:62
- Mate:595: motor_mount:1 ↔ AS 1112 (2) - Metric M2  Type 5:62
- Mate:596: motor_mount:4 ↔ AS 1112 (2) - Metric M2  Type 5:60
- Mate:597: motor_mount:4 ↔ AS 1112 (2) - Metric M2  Type 5:60
- Mate:598: motor_mount:4 ↔ AS 1112 (2) - Metric M2  Type 5:59
- Mate:599: motor_mount:4 ↔ AS 1112 (2) - Metric M2  Type 5:59
- Mate:600: motor_mount:3 ↔ AS 1112 (2) - Metric M2  Type 5:57
- Mate:601: motor_mount:3 ↔ AS 1112 (2) - Metric M2  Type 5:57
- Mate:602: motor_mount:3 ↔ AS 1112 (2) - Metric M2  Type 5:58
- Mate:603: motor_mount:3 ↔ AS 1112 (2) - Metric M2  Type 5:58
- Mate:604: motor_mount_lock:3 ↔ AS 1427 H - Metric M2 x 12:1
- Mate:605: motor_mount_lock:3 ↔ AS 1427 H - Metric M2 x 12:1
- Mate:606: motor_mount_lock:3 ↔ AS 1427 H - Metric M2 x 12:2
- Mate:607: motor_mount_lock:3 ↔ AS 1427 H - Metric M2 x 12:2
- Mate:608: motor_mount_lock:4 ↔ AS 1427 H - Metric M2 x 12:5
- Mate:609: motor_mount_lock:4 ↔ AS 1427 H - Metric M2 x 12:5
- Mate:610: motor_mount_lock:4 ↔ AS 1427 H - Metric M2 x 12:6
- Mate:611: motor_mount_lock:4 ↔ AS 1427 H - Metric M2 x 12:6
- Mate:612: motor_mount_lock:1 ↔ AS 1427 H - Metric M2 x 12:8
- Mate:613: motor_mount_lock:1 ↔ AS 1427 H - Metric M2 x 12:8
- Mate:614: motor_mount_lock:1 ↔ AS 1427 H - Metric M2 x 12:7
- Mate:615: motor_mount_lock:1 ↔ AS 1427 H - Metric M2 x 12:7
- Mate:616: motor_mount_lock:2 ↔ AS 1427 H - Metric M2 x 12:3
- Mate:617: motor_mount_lock:2 ↔ AS 1427 H - Metric M2 x 12:3
- Mate:618: motor_mount_lock:2 ↔ AS 1427 H - Metric M2 x 12:4
- Mate:619: motor_mount_lock:2 ↔ AS 1427 H - Metric M2 x 12:4
- Mate:620: motor_mount_lock:2 ↔ AS 1427 H - Metric M3 x 10:1
- Mate:621: motor_mount_lock:2 ↔ AS 1427 H - Metric M3 x 10:1
- Mate:622: arm_front_rect:1 ↔ ANSI B18.2.4.2M M3x0,5:1
- Mate:623: AS 1427 H - Metric M3 x 10:1 ↔ ANSI B18.2.4.2M M3x0,5:1
- Mate:624: motor_mount_lock:3 ↔ AS 1427 H - Metric M3 x 10:2
- Mate:625: motor_mount_lock:3 ↔ AS 1427 H - Metric M3 x 10:2
- Mate:626: motor_mount_lock:4 ↔ AS 1427 H - Metric M3 x 10:3
- Mate:627: motor_mount_lock:4 ↔ AS 1427 H - Metric M3 x 10:3
- Mate:628: motor_mount_lock:1 ↔ AS 1427 H - Metric M3 x 10:4
- Mate:629: motor_mount_lock:1 ↔ AS 1427 H - Metric M3 x 10:4
- Mate:630: arm_back_rect:1 ↔ ANSI B18.2.4.2M M3x0,5:2
- Mate:631: AS 1427 H - Metric M3 x 10:2 ↔ ANSI B18.2.4.2M M3x0,5:2
- Mate:632: arm_back_rect:2 ↔ ANSI B18.2.4.2M M3x0,5:3
- Mate:633: AS 1427 H - Metric M3 x 10:3 ↔ ANSI B18.2.4.2M M3x0,5:3